# Autodesk Inventor assembly: CamLeftNCS
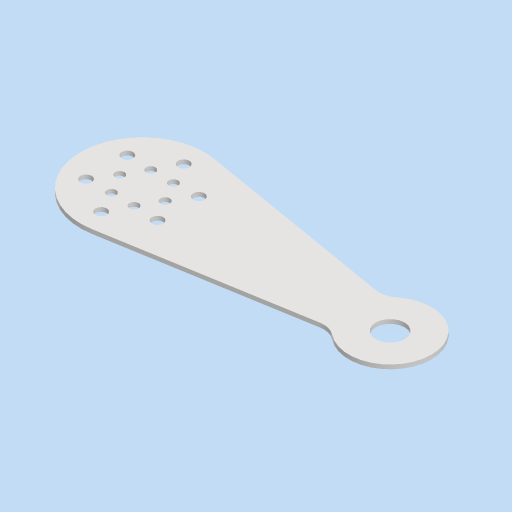
[picture p0: Inventor's stored thumbnail of the model, 512x512]
Saved by Autodesk Inventor 2023 (Build 270158000, 158)
## iProperties
Created: 2026-06-18
Part Number: CamLeftNCS
Document SubType Name: Assembly
Designer: Nathann
Author: Nathann
## Documents named in this file (2)
- C:\Users\Nathann\ClawdDrive\Objet3D\RunningRobot\PartURDF\CamLeftNCS.iam
- C:\Users\Nathann\ClawdDrive\Objet3D\RunningRobot\PartURDF\CamLeft_Simplify_1.ipt
## Components (1 placed, 1 different names)
1. CamLeft_Simplify_1:1 — Mate:1, Flush:1, Mate:2
## Relationships (4: Mate 3, Flush 1)
- Mate:1: CamLeft_Simplify_1:1
- Flush:1: CamLeft_Simplify_1:1
- Mate:2: CamLeft_Simplify_1:1
- Mate:3
